# Autodesk Inventor assembly: 0002_Tam_nguyen_Truc_Z
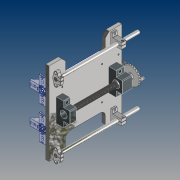
[picture p0: Inventor's stored thumbnail of the model, 180x180]
Saved by Autodesk Inventor 2021 (Build 250183000, 183)
## iProperties
Created: 2024-04-08
Part Number: 0002_Tam_nguyen_Truc_Z
Document SubType Name: Assembly
Designer: Admin
Mass: 5555.42 g
Surface Area: 1871.93 cm^2
Volume: 729.133 cm^3
Density: 7.61921 g/cm^3
Author: Admin
## Documents named in this file (13)
- C:\Users\Admin\Desktop\DO_AN_TOT_NGHIEP_2024\Mechanical\Design_in_3D\Version_2\0002_Tam_nguyen_Truc_Z.iam
- C:\Users\Admin\Desktop\DO_AN_TOT_NGHIEP_2024\Mechanical\Design_in_3D\Version_2\0002_Truc_Z.iam
- C:\Users\Admin\Desktop\DO_AN_TOT_NGHIEP_2024\Mechanical\Design_in_3D\Version_2\08_Tam_truc_Z.ipt
- C:\Users\Admin\Desktop\DO_AN_TOT_NGHIEP_2024\Mechanical\Design_in_3D\Library\sk10-3.snapshot.2\SK10.ipt
- C:\Users\Admin\Desktop\DO_AN_TOT_NGHIEP_2024\Mechanical\Design_in_3D\Version_2\09_Truc_song_song_x10x250.ipt
- C:\Users\Admin\Desktop\DO_AN_TOT_NGHIEP_2024\Mechanical\Design_in_3D\Library\shf10-shf8-linear-shaft-support-1.snapshot.6\SHF8.ipt
- C:\Users\Admin\Desktop\DO_AN_TOT_NGHIEP_2024\Mechanical\Design_in_3D\Library\ke-goc-vuong-nhom-2020-ke-n-i-1.snapshot.1\ke-nhom-noi-2020.ipt
- C:\Users\Admin\Desktop\DO_AN_TOT_NGHIEP_2024\Mechanical\Design_in_3D\Library\khung-nhom-d-nh-hinh-trong-cong-nghi-p-1.snapshot.1\Modify_Ky_Anh\20x20x200.ipt
- C:\Users\Admin\Desktop\DO_AN_TOT_NGHIEP_2024\Mechanical\Design_in_3D\Version_2\10_Banh_lai.ipt
- C:\Users\Admin\Desktop\DO_AN_TOT_NGHIEP_2024\Mechanical\Design_in_3D\Version_2\11_Chot_banh_lai.ipt
- C:\Users\Admin\Documents\Inventor\Content Center Files\R2021\en-US\BS EN ISO 4762\BS EN ISO 4762 - M4 x 25(1).ipt
- C:\Users\Admin\Desktop\DO_AN_TOT_NGHIEP_2024\Mechanical\Design_in_3D\Library\Lo_xo_phi_7x40.ipt
- C:\Users\Admin\Documents\Inventor\Content Center Files\R2021\en-US\AS 1237 (D1)\AS 1237 - 6 mm(5).ipt
## Components (23 placed, 12 different names)
1. 0002_Truc_Z:1 [sub-assembly] — Mate:1, Mate:2, Angle:1, Mate:5, Flush:7, Mate:10, Mate:24
2. 08_Tam_truc_Z:1 — Mate:1, Mate:2, Mate:3, Mate:4, Angle:2, Flush:6, Flush:7, Mate:11, Mate:12, Flush:8, Flush:9, Mate:13, Mate:15, Flush:10, Mate:17
3. SK10:1 — Mate:3, Flush:1, Mate:5, Mate:6
4. SK10:2 — Mate:4, Angle:1, Flush:1, Mate:7, Mate:23
5. 09_Truc_song_song_x10x250:1 — Mate:7, Flush:2, Mate:8, Flush:5, Mate:10
6. 09_Truc_song_song_x10x250:2 — Mate:6, Flush:2, Mate:9
7. SHF8:1 — Flush:3, Mate:8, Angle:2, Flush:4, Flush:5, Flush:6
8. SHF8:2 — Flush:3, Mate:9, Flush:4
9. ke-nhom-noi-2020:1 — Mate:16, Flush:11, Flush:12
10. 20x20x200:1 — Mate:11, Flush:9, Symmetry:1, Flush:10, Mate:16, Flush:11, Flush:12, Flush:13, Mate:18, Flush:14, Flush:15, Mate:19
11. 20x20x200:2 — Mate:12, Flush:8, Mate:14, Symmetry:1, Mate:20, Flush:16, Flush:17, Mate:21, Flush:18, Flush:19, Flush:20, Mate:22, Flush:21
12. 20x20x200:3 — Mate:13, Mate:14, Mate:15, Mate:23, Mate:27, Mate:28
13. ke-nhom-noi-2020:2 — Mate:18, Flush:14, Flush:15
14. ke-nhom-noi-2020:3 — Mate:20, Flush:16, Flush:17
15. ke-nhom-noi-2020:4 — Flush:20, Mate:22, Flush:21
16. ke-nhom-noi-2020:5 — Mate:21, Flush:18, Flush:19
17. ke-nhom-noi-2020:6 — Mate:17, Flush:13, Mate:19
18. 10_Banh_lai:1 — Mate:24, Mate:26
19. 11_Chot_banh_lai:1 — Mate:26, Mate:27, Mate:28, Mate:29, Mate:32, Insert:1
20. BS EN ISO 4762 - Metric M4 x 25:1 — Mate:29, Mate:30, Mate:31, Mate:33, Mate:34
21. Lo_xo_phi_7x40:1 — Mate:30, Mate:31, Mate:32
22. AS 1237 (D1) 6 mm:1 — Mate:33, Mate:34
23. AS 1237 (D1) 6 mm:2 — Insert:1
## Relationships (58: Mate 33, Flush 21, Angle 2, Symmetry 1, Insert 1)
- Mate:1: 0002_Truc_Z:1 ↔ 08_Tam_truc_Z:1
- Mate:2: 0002_Truc_Z:1 ↔ 08_Tam_truc_Z:1
- Mate:3: 08_Tam_truc_Z:1 ↔ SK10:1
- Mate:4: 08_Tam_truc_Z:1 ↔ SK10:2
- Angle:1 (0 deg): 0002_Truc_Z:1 ↔ SK10:2
- Flush:1: SK10:1 ↔ SK10:2
- Mate:5 (100 mm): 0002_Truc_Z:1 ↔ SK10:1
- Mate:6: SK10:1 ↔ 09_Truc_song_song_x10x250:2
- Mate:7: SK10:2 ↔ 09_Truc_song_song_x10x250:1
- Flush:2: 09_Truc_song_song_x10x250:1 ↔ 09_Truc_song_song_x10x250:2
- Flush:3: SHF8:1 ↔ SHF8:2
- Mate:8: 09_Truc_song_song_x10x250:1 ↔ SHF8:1
- Angle:2 (0 deg): 08_Tam_truc_Z:1 ↔ SHF8:1
- Mate:9: 09_Truc_song_song_x10x250:2 ↔ SHF8:2
- Flush:4: SHF8:1 ↔ SHF8:2
- Flush:5: 09_Truc_song_song_x10x250:1 ↔ SHF8:1
- Flush:6: 08_Tam_truc_Z:1 ↔ SHF8:1
- Flush:7 (20 mm): 0002_Truc_Z:1 ↔ 08_Tam_truc_Z:1
- Mate:10 (100 mm): 0002_Truc_Z:1 ↔ 09_Truc_song_song_x10x250:1
- Mate:11: 08_Tam_truc_Z:1 ↔ 20x20x200:1
- Mate:12: 08_Tam_truc_Z:1 ↔ 20x20x200:2
- Flush:8: 08_Tam_truc_Z:1 ↔ 20x20x200:2
- Flush:9: 08_Tam_truc_Z:1 ↔ 20x20x200:1
- Mate:13: 08_Tam_truc_Z:1 ↔ 20x20x200:3
- Mate:14: 20x20x200:2 ↔ 20x20x200:3
- Mate:15: 08_Tam_truc_Z:1 ↔ 20x20x200:3
- Symmetry:1: 20x20x200:1 ↔ 20x20x200:2
- Flush:10 (65 mm): 08_Tam_truc_Z:1 ↔ 20x20x200:1
- Mate:16: ke-nhom-noi-2020:1 ↔ 20x20x200:1
- Flush:11 (0.242 mm): ke-nhom-noi-2020:1 ↔ 20x20x200:1
- Flush:12: ke-nhom-noi-2020:1 ↔ 20x20x200:1
- Mate:17: 08_Tam_truc_Z:1 ↔ ke-nhom-noi-2020:6
- Flush:13: 20x20x200:1 ↔ ke-nhom-noi-2020:6
- Mate:18: 20x20x200:1 ↔ ke-nhom-noi-2020:2
- Flush:14: 20x20x200:1 ↔ ke-nhom-noi-2020:2
- Flush:15: 20x20x200:1 ↔ ke-nhom-noi-2020:2
- Mate:19: 20x20x200:1 ↔ ke-nhom-noi-2020:6
- Mate:20: 20x20x200:2 ↔ ke-nhom-noi-2020:3
- Flush:16: 20x20x200:2 ↔ ke-nhom-noi-2020:3
- Flush:17: 20x20x200:2 ↔ ke-nhom-noi-2020:3
- Mate:21: 20x20x200:2 ↔ ke-nhom-noi-2020:5
- Flush:18: 20x20x200:2 ↔ ke-nhom-noi-2020:5
- Flush:19: 20x20x200:2 ↔ ke-nhom-noi-2020:5
- Flush:20: 20x20x200:2 ↔ ke-nhom-noi-2020:4
- Mate:22: 20x20x200:2 ↔ ke-nhom-noi-2020:4
- Flush:21: 20x20x200:2 ↔ ke-nhom-noi-2020:4
- Mate:23: SK10:2 ↔ 20x20x200:3
- Mate:24: 0002_Truc_Z:1 ↔ 10_Banh_lai:1
- Mate:26: 10_Banh_lai:1 ↔ 11_Chot_banh_lai:1
- Mate:27: 20x20x200:3 ↔ 11_Chot_banh_lai:1
- Mate:28: 20x20x200:3 ↔ 11_Chot_banh_lai:1
- Mate:29: 11_Chot_banh_lai:1 ↔ BS EN ISO 4762 - Metric M4 x 25:1
- Mate:30: BS EN ISO 4762 - Metric M4 x 25:1 ↔ Lo_xo_phi_7x40:1
- Mate:31: BS EN ISO 4762 - Metric M4 x 25:1 ↔ Lo_xo_phi_7x40:1
- Mate:32: 11_Chot_banh_lai:1 ↔ Lo_xo_phi_7x40:1
- Mate:33: BS EN ISO 4762 - Metric M4 x 25:1 ↔ AS 1237 (D1) 6 mm:1
- Mate:34: BS EN ISO 4762 - Metric M4 x 25:1 ↔ AS 1237 (D1) 6 mm:1
- Insert:1: 11_Chot_banh_lai:1 ↔ AS 1237 (D1) 6 mm:2
